# Autodesk Inventor assembly: MotorFufuPounder
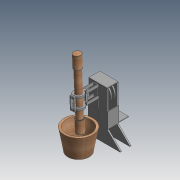
[picture p0: Inventor's stored thumbnail of the model, 180x180]
Saved by Autodesk Inventor 2015 (Build 190159000, 159)
## iProperties
Created: 2014-08-31
Part Number: MotorFufuPounder
Document SubType Name: Assembly
Designer: shohei
Author: shohei
## Documents named in this file (4)
- C:\Users\shohei\Documents\Inventor\FufuPounderGeared\MotorFufuPounder.iam
- C:\Users\shohei\Documents\Inventor\FufuPounderGeared\rev6.iam
- C:\Users\shohei\Documents\Inventor\FufuPounderGeared\GearAssembly_rev1.iam
- C:\Users\shohei\Documents\Inventor\FufuPounderGeared\guardplate.ipt
## Components (4 placed, 3 different names)
1. rev6:1 [sub-assembly] — Flush:1, Mate:1, Flush:2, Mate:2, Flush:3
2. GearAssembly_rev1:1 [sub-assembly] — Flush:1
3. guardplate:1 — Mate:1, Flush:2
4. guardplate:2 — Mate:2, Flush:3
## Relationships (5: Flush 3, Mate 2)
- Flush:1: rev6:1 ↔ GearAssembly_rev1:1
- Mate:1: rev6:1 ↔ guardplate:1
- Flush:2: rev6:1 ↔ guardplate:1
- Mate:2: rev6:1 ↔ guardplate:2
- Flush:3: rev6:1 ↔ guardplate:2
